# Autodesk Inventor assembly: Crankshaft Subassembly
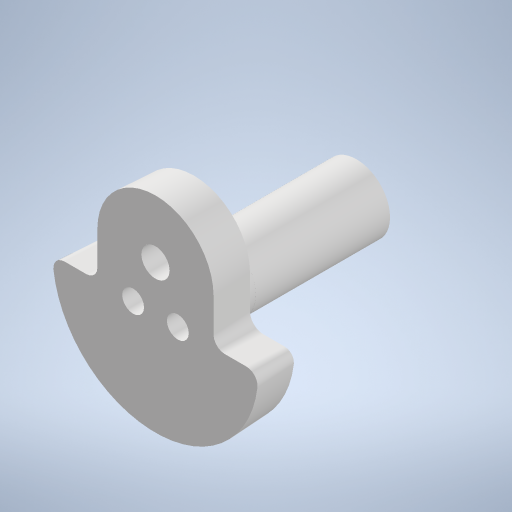
[picture p0: Inventor's stored thumbnail of the model, 512x512]
Saved by Autodesk Inventor 2023 (Build 270158000, 158)
## iProperties
Created: 2022-12-25
Part Number: Crankshaft Subassembly
Document SubType Name: Assembly
Designer: tgr41
Author: tgr41
## Documents named in this file (3)
- C:\Users\tgr41\OneDrive\Documents\Repositories\Steam-Engine\2 Inch V3\Crankshaft Subassembly.iam
- C:\Users\tgr41\OneDrive\Documents\Repositories\Steam-Engine\2 Inch V3\Crank on Crankshaft.ipt
- C:\Users\tgr41\OneDrive\Documents\Repositories\Steam-Engine\2 Inch V3\Crankshaft.ipt
## Components (2 placed, 2 different names)
1. Crank on Crankshaft:1 — Mate:1, Mate:2, Mate:3
2. Crankshaft:1 — Mate:1, Mate:2, Mate:3
## Relationships (3: Mate 3)
- Mate:1: Crank on Crankshaft:1 ↔ Crankshaft:1
- Mate:2: Crank on Crankshaft:1 ↔ Crankshaft:1
- Mate:3: Crank on Crankshaft:1 ↔ Crankshaft:1
